# Autodesk Inventor assembly: Full Rack
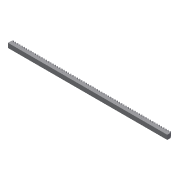
[picture p0: Inventor's stored thumbnail of the model, 180x180]
Saved by Autodesk Inventor 2016 (Build 200138000, 138)
## iProperties
Created: 2016-04-05
Part Number: Full Rack
Document SubType Name: Assembly
Designer: Ariana
Author: Ariana
## Documents named in this file (2)
- C:\Users\Ariana\Downloads\Capstone CAD\Capstone CAD\Delivery\Full Rack.iam
- C:\Users\Ariana\Downloads\Capstone CAD\Capstone CAD\Delivery\Rack.ipt
## Components (6 placed, 1 different names)
1. Rack:1 — Mate:1, Flush:1, Flush:2
2. Rack:2 — Mate:5, Flush:7, Flush:10
3. Rack:3 — Mate:1, Flush:1, Flush:2, Flush:3, Flush:4, Mate:2
4. Rack:4 — Mate:3, Mate:4, Flush:5, Flush:6, Flush:8, Flush:9
5. Rack:5 — Mate:4, Mate:5, Flush:6, Flush:7, Flush:9, Flush:10
6. Rack:6 — Flush:3, Flush:4, Mate:2, Mate:3, Flush:5, Flush:8
## Relationships (15: Flush 10, Mate 5)
- Mate:1: Rack:1 ↔ Rack:3
- Flush:1: Rack:1 ↔ Rack:3
- Flush:2: Rack:1 ↔ Rack:3
- Flush:3: Rack:3 ↔ Rack:6
- Flush:4: Rack:3 ↔ Rack:6
- Mate:2: Rack:3 ↔ Rack:6
- Mate:3: Rack:4 ↔ Rack:6
- Mate:4: Rack:4 ↔ Rack:5
- Mate:5: Rack:2 ↔ Rack:5
- Flush:5: Rack:4 ↔ Rack:6
- Flush:6: Rack:4 ↔ Rack:5
- Flush:7: Rack:2 ↔ Rack:5
- Flush:8: Rack:4 ↔ Rack:6
- Flush:9: Rack:4 ↔ Rack:5
- Flush:10: Rack:2 ↔ Rack:5
